# Autodesk Inventor assembly: ASM Heating Unit
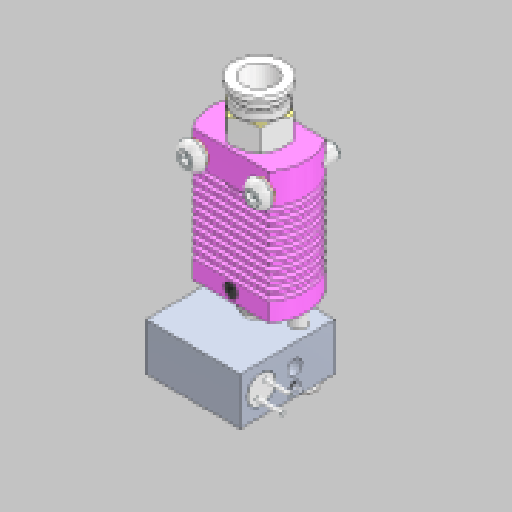
[picture p0: Inventor's stored thumbnail of the model, 512x512]
Saved by Autodesk Inventor 2025.4 (Build 294407000, 407)
## iProperties
Created: 2026-03-02
Part Number: ASM Heating Unit
Document SubType Name: Assembly
Designer: Inema
Author: Inema
Revision Number: ANY
## Documents named in this file (12)
- C:\Users\Inema\OneDrive\GitHub\Ender-3\Ender-3 Mechanical\Modificada\Extrusor Original\ASM Heating Unit.iam
- C:\Users\Inema\OneDrive\GitHub\Ender-3\Ender-3 Mechanical\Modificada\Extrusor Original\Radiator.ipt
- C:\Users\Inema\OneDrive\GitHub\Ender-3\Ender-3 Mechanical\Modificada\Extrusor Original\nozzle.ipt
- C:\Users\Inema\OneDrive\GitHub\Ender-3\Ender-3 Mechanical\Modificada\Extrusor Original\Heat block.ipt
- C:\Users\Inema\OneDrive\GitHub\Ender-3\Ender-3 Mechanical\Modificada\Extrusor Original\Pneumatic joint.ipt
- C:\Users\Inema\OneDrive\GitHub\Ender-3\Ender-3 Mechanical\Modificada\Extrusor Original\Nozzle thermistor.ipt
- C:\Users\Inema\OneDrive\GitHub\Ender-3\Ender-3 Mechanical\Modificada\Extrusor Original\Heater.ipt
- C:\Users\Inema\OneDrive\GitHub\Ender-3\Ender-3 Mechanical\Modificada\Extrusor Original\M3X16 Pan Head Screw.ipt
- C:\Users\Inema\OneDrive\GitHub\Ender-3\Ender-3 Mechanical\Modificada\Extrusor Original\M3 Split Washer.ipt
- C:\Users\Inema\OneDrive\GitHub\Ender-3\Ender-3 Mechanical\Modificada\Extrusor Original\M3×18 Flush Head Screw.ipt
- C:\Users\Inema\OneDrive\GitHub\Ender-3\Ender-3 Mechanical\Modificada\Extrusor Original\M3 Screw.ipt
- C:\Users\Inema\OneDrive\GitHub\Ender-3\Ender-3 Mechanical\Modificada\HeatBreak.ipt
## Components (15 placed, 15 different names)
1. Radiator_200 — Coincidencia:1, Coincidencia:2, Coincidencia:3, Coincidencia:4, Insertar:5
2. nozzle_201 — Insertar:1, Coincidencia:6
3. Heat block_202 — Insertar:1, Coincidencia:5, Insertar:2, Insertar:3, Insertar:4, Coincidencia:7, Insertar:6
4. Pneumatic joint_203
5. Nozzle thermistor_204 — Coincidencia:7
6. Heater_205 — Insertar:4
7. M3X16 Pan Head Screw_206 — Insertar:7
8. M3 Split Washer_207 — Insertar:7
9. M3×18 Flush Head Screw_208 — Coincidencia:1, Insertar:2
10. M3×18 Flush Head Screw_209 — Coincidencia:2, Insertar:3
11. M3 Screw_210 — Insertar:6
12. M3X16 Pan Head Screw_211 — Insertar:8
13. M3 Split Washer_212 — Insertar:8
14. M3 Screw_213 — Insertar:5
15. HeatBreak:1 — Coincidencia:3, Coincidencia:4, Coincidencia:5, Coincidencia:6
## Relationships (15: Insert 8, Mate 7)
- Coincidencia:1 [Mate]: Radiator_200 ↔ M3×18 Flush Head Screw_208
- Coincidencia:2 [Mate]: Radiator_200 ↔ M3×18 Flush Head Screw_209
- Insertar:1 (1 mm): nozzle_201 ↔ Heat block_202
- Coincidencia:3 [Mate]: Radiator_200 ↔ HeatBreak:1
- Coincidencia:4 [Mate]: Radiator_200 ↔ HeatBreak:1
- Coincidencia:5 [Mate]: Heat block_202 ↔ HeatBreak:1
- Coincidencia:6 [Mate]: nozzle_201 ↔ HeatBreak:1
- Insertar:2: Heat block_202 ↔ M3×18 Flush Head Screw_208
- Insertar:3: Heat block_202 ↔ M3×18 Flush Head Screw_209
- Insertar:4: Heat block_202 ↔ Heater_205
- Insertar:5: Radiator_200 ↔ M3 Screw_213
- Coincidencia:7 [Mate]: Heat block_202 ↔ Nozzle thermistor_204
- Insertar:6: Heat block_202 ↔ M3 Screw_210
- Insertar:7: M3X16 Pan Head Screw_206 ↔ M3 Split Washer_207
- Insertar:8: M3X16 Pan Head Screw_211 ↔ M3 Split Washer_212
